# Autodesk Inventor assembly: złożenie przekładni
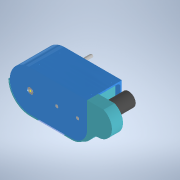
[picture p0: Inventor's stored thumbnail of the model, 180x180]
Saved by Autodesk Inventor 2021 (Build 250183000, 183)
## iProperties
Created: 2021-06-25
Part Number: złożenie przekładni
Document SubType Name: Assembly
Designer: Łukasz
Author: Łukasz
## Documents named in this file (17)
- E:\GITHUB_Czołg\Szybki-Czolg-antyRadziecki\złożenie przekładni.iam
- E:\GITHUB_Czołg\Szybki-Czolg-antyRadziecki\obudowa przekładni.ipt
- C:\Users\Łukasz\Documents\Inventor\Content Center Files\R2021\en-US\BS 292 (I)\BS 292 Part 1 - 608 - 8 x 22 x 7.ipt
- E:\GITHUB_Czołg\Szybki-Czolg-antyRadziecki\oś napędowa.ipt
- E:\GITHUB_Czołg\Szybki-Czolg-antyRadziecki\oś 8mm x 91mm.ipt
- E:\GITHUB_Czołg\Szybki-Czolg-antyRadziecki\koła zębate\Design Accelerator\inny set zebow\Design Accelerator\Spur Gear11.ipt
- E:\GITHUB_Czołg\Szybki-Czolg-antyRadziecki\koła zębate\Design Accelerator\podwojne koło zebate.iam
- E:\GITHUB_Czołg\Szybki-Czolg-antyRadziecki\koła zębate\Design Accelerator\podwojne koło zebate drugi skręt.iam
- E:\GITHUB_Czołg\Szybki-Czolg-antyRadziecki\koła zębate\Design Accelerator\inny set zebow\Design Accelerator\napędowy 40 zębow.ipt
- E:\GITHUB_Czołg\Szybki-Czolg-antyRadziecki\inne zęby\Design Accelerator\Spur Gear22.ipt
- E:\GITHUB_Czołg\Szybki-Czolg-antyRadziecki\silnik 3660.ipt
- E:\GITHUB_Czołg\Szybki-Czolg-antyRadziecki\koła zębate\Design Accelerator\inny set zebow\Design Accelerator\Spur Gear11 motor.ipt
- E:\GITHUB_Czołg\Szybki-Czolg-antyRadziecki\obudowa przekładni 2.ipt
- E:\GITHUB_Czołg\Szybki-Czolg-antyRadziecki\obudowa przekładni 3.ipt
- E:\GITHUB_Czołg\Szybki-Czolg-antyRadziecki\obudowa przekładni 4.ipt
- E:\GITHUB_Czołg\Szybki-Czolg-antyRadziecki\obudowa przekładni 5.ipt
- E:\GITHUB_Czołg\Szybki-Czolg-antyRadziecki\obudowa przekładni 6.ipt
## Components (30 placed, 14 different names)
1. obudowa przekładni:1 — Rotational:14, Rotational:15, Rigid:16, Rotational:16, Rotational:17, Rotational:18, Flush:2, Mate:1, Mate:2, Flush:3, Mate:3, Mate:4, Flush:6, Mate:6, Flush:7, Mate:8, Flush:8, Mate:10
2. BS 292: Part 1 (I) (Metric) 608 - 8 x 22 x 7:2 — Rotational:3, Rotational:5, Rotational:15
3. BS 292: Part 1 (I) (Metric) 608 - 8 x 22 x 7:1 — Rotational:14
4. oś napędowa:1 — Rotational:3, Rigid:15
5. oś 8mm x 91mm:1 — Rigid:16
6. Spur Gear1:1 — Rotational:4, Rotation:1, Rotational:7, Rotation:6, Rotational:17
7. podwojne koło zebate:1 [sub-assembly] — Rigid:4, Rigid:5, Rotation:1, Rotation:2
8. podwojne koło zebate:3 [sub-assembly] — Rigid:8, Rigid:9, Rotation:3, Rotation:4
9. BS 292: Part 1 (I) (Metric) 608 - 8 x 22 x 7:3 — Rotational:4
10. BS 292: Part 1 (I) (Metric) 608 - 8 x 22 x 7:4 — Rigid:4, Rotational:5
11. BS 292: Part 1 (I) (Metric) 608 - 8 x 22 x 7:5 — Rigid:5, Rotational:8
12. BS 292: Part 1 (I) (Metric) 608 - 8 x 22 x 7:6 — Rotational:7, Rotational:9
13. BS 292: Part 1 (I) (Metric) 608 - 8 x 22 x 7:7 — Rigid:12, Rotational:10
14. BS 292: Part 1 (I) (Metric) 608 - 8 x 22 x 7:8 — Rigid:8, Rotational:8
15. BS 292: Part 1 (I) (Metric) 608 - 8 x 22 x 7:9 — Rigid:9
16. BS 292: Part 1 (I) (Metric) 608 - 8 x 22 x 7:10 — Rigid:13, Rotational:10
17. BS 292: Part 1 (I) (Metric) 608 - 8 x 22 x 7:11 — Rigid:14
18. podwojne koło zebate drugi skręt:1 [sub-assembly] — Rigid:12, Rotational:9, Rotation:2, Rotation:3
19. podwojne koło zebate drugi skręt:2 [sub-assembly] — Rigid:13, Rigid:14, Rotation:4, Rotation:5
20. Spur Gear2:1 — Rigid:15, Rotation:5
21. oś 8mm x 91mm:2 — Rotational:16
22. Spur Gear2:2 — Rotational:11, Rotation:6, Flush:1, Tangent:1, Rotational:18, obrot silnika
23. BS 292: Part 1 (I) (Metric) 608 - 8 x 22 x 7:12 — Rotational:11
24. silnik 3660:1 — Flush:1, Tangent:1, Rotational:19
25. Spur Gear1:2 — Rotational:19, obrot silnika
26. obudowa przekładni 2:1 — Flush:2, Mate:1, Mate:2
27. obudowa przekładni 3:1 — Flush:3, Mate:3, Mate:4, Mate:7, Flush:9, Mate:9
28. obudowa przekładni 4:1 — Flush:6, Mate:6, Mate:7
29. obudowa przekładni 5:1 — Flush:7, Mate:8, Flush:8
30. obudowa przekładni 6:1 — Flush:9, Mate:9, Mate:10
## Relationships (47: RevoluteJoint 14, WeldJoint 9, Mate 9, RelateRotation 7, Flush 7, Tangent 1)
- Rotational:3 [RevoluteJoint]: BS 292: Part 1 (I) (Metric) 608 - 8 x 22 x 7:2 ↔ oś napędowa:1
- Rotational:4 [RevoluteJoint] (-3.5 mm): Spur Gear1:1 ↔ BS 292: Part 1 (I) (Metric) 608 - 8 x 22 x 7:3
- Rigid:4 [WeldJoint]: podwojne koło zebate:1 ↔ BS 292: Part 1 (I) (Metric) 608 - 8 x 22 x 7:4
- Rigid:5 [WeldJoint]: podwojne koło zebate:1 ↔ BS 292: Part 1 (I) (Metric) 608 - 8 x 22 x 7:5
- Rigid:8 [WeldJoint]: podwojne koło zebate:3 ↔ BS 292: Part 1 (I) (Metric) 608 - 8 x 22 x 7:8
- Rigid:9 [WeldJoint]: podwojne koło zebate:3 ↔ BS 292: Part 1 (I) (Metric) 608 - 8 x 22 x 7:9
- Rotational:5 [RevoluteJoint] (2 mm): BS 292: Part 1 (I) (Metric) 608 - 8 x 22 x 7:2 ↔ BS 292: Part 1 (I) (Metric) 608 - 8 x 22 x 7:4
- Rotation:1 [RelateRotation] (2 ul): Spur Gear1:1 ↔ podwojne koło zebate:1
- Rotational:7 [RevoluteJoint] (-2 mm): Spur Gear1:1 ↔ BS 292: Part 1 (I) (Metric) 608 - 8 x 22 x 7:6
- Rotational:8 [RevoluteJoint] (2 mm): BS 292: Part 1 (I) (Metric) 608 - 8 x 22 x 7:5 ↔ BS 292: Part 1 (I) (Metric) 608 - 8 x 22 x 7:8
- Rigid:12 [WeldJoint]: BS 292: Part 1 (I) (Metric) 608 - 8 x 22 x 7:7 ↔ podwojne koło zebate drugi skręt:1
- Rotational:9 [RevoluteJoint]: BS 292: Part 1 (I) (Metric) 608 - 8 x 22 x 7:6 ↔ podwojne koło zebate drugi skręt:1
- Rotation:2 [RelateRotation] (2 ul): podwojne koło zebate:1 ↔ podwojne koło zebate drugi skręt:1
- Rotation:3 [RelateRotation] (2 ul): podwojne koło zebate:3 ↔ podwojne koło zebate drugi skręt:1
- Rigid:13 [WeldJoint]: BS 292: Part 1 (I) (Metric) 608 - 8 x 22 x 7:10 ↔ podwojne koło zebate drugi skręt:2
- Rigid:14 [WeldJoint]: BS 292: Part 1 (I) (Metric) 608 - 8 x 22 x 7:11 ↔ podwojne koło zebate drugi skręt:2
- Rotational:10 [RevoluteJoint] (2 mm): BS 292: Part 1 (I) (Metric) 608 - 8 x 22 x 7:7 ↔ BS 292: Part 1 (I) (Metric) 608 - 8 x 22 x 7:10
- Rotation:4 [RelateRotation] (2 ul): podwojne koło zebate:3 ↔ podwojne koło zebate drugi skręt:2
- Rigid:15 [WeldJoint] (-23 mm): oś napędowa:1 ↔ Spur Gear2:1
- Rotation:5 [RelateRotation] (2 ul): podwojne koło zebate drugi skręt:2 ↔ Spur Gear2:1
- Rotational:11 [RevoluteJoint] (-1 mm): Spur Gear2:2 ↔ BS 292: Part 1 (I) (Metric) 608 - 8 x 22 x 7:12
- Rotation:6 [RelateRotation] (1.35 ul): Spur Gear1:1 ↔ Spur Gear2:2
- Flush:1 (16 mm): Spur Gear2:2 ↔ silnik 3660:1
- Tangent:1 (25 mm): Spur Gear2:2 ↔ silnik 3660:1
- Rotational:14 [RevoluteJoint]: obudowa przekładni:1 ↔ BS 292: Part 1 (I) (Metric) 608 - 8 x 22 x 7:1
- Rotational:15 [RevoluteJoint]: obudowa przekładni:1 ↔ BS 292: Part 1 (I) (Metric) 608 - 8 x 22 x 7:2
- Rigid:16 [WeldJoint]: obudowa przekładni:1 ↔ oś 8mm x 91mm:1
- Rotational:16 [RevoluteJoint]: obudowa przekładni:1 ↔ oś 8mm x 91mm:2
- Rotational:17 [RevoluteJoint] (2 mm): obudowa przekładni:1 ↔ Spur Gear1:1
- Rotational:18 [RevoluteJoint] (2 mm): obudowa przekładni:1 ↔ Spur Gear2:2
- Rotational:19 [RevoluteJoint]: silnik 3660:1 ↔ Spur Gear1:2
- obrot silnika [RelateRotation] (1.35 ul): Spur Gear2:2 ↔ Spur Gear1:2
- Flush:2: obudowa przekładni:1 ↔ obudowa przekładni 2:1
- Mate:1: obudowa przekładni:1 ↔ obudowa przekładni 2:1
- Mate:2: obudowa przekładni:1 ↔ obudowa przekładni 2:1
- Flush:3: obudowa przekładni:1 ↔ obudowa przekładni 3:1
- Mate:3: obudowa przekładni:1 ↔ obudowa przekładni 3:1
- Mate:4: obudowa przekładni:1 ↔ obudowa przekładni 3:1
- Flush:6: obudowa przekładni:1 ↔ obudowa przekładni 4:1
- Mate:6: obudowa przekładni:1 ↔ obudowa przekładni 4:1
- Mate:7: obudowa przekładni 3:1 ↔ obudowa przekładni 4:1
- Flush:7: obudowa przekładni:1 ↔ obudowa przekładni 5:1
- Mate:8: obudowa przekładni:1 ↔ obudowa przekładni 5:1
- Flush:8: obudowa przekładni:1 ↔ obudowa przekładni 5:1
- Flush:9: obudowa przekładni 3:1 ↔ obudowa przekładni 6:1
- Mate:9: obudowa przekładni 3:1 ↔ obudowa przekładni 6:1
- Mate:10: obudowa przekładni:1 ↔ obudowa przekładni 6:1
